# Autodesk Inventor assembly: Assembled
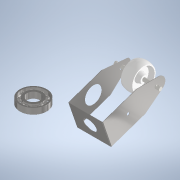
[picture p0: Inventor's stored thumbnail of the model, 180x180]
Saved by Autodesk Inventor 2020.3 (Build 243373000, 373)
## iProperties
Created: 2022-06-27
Part Number: Assembled
Document SubType Name: Assembly
Designer: 0x6f736f646f
Author: 0x6f736f646f
## Documents named in this file (5)
- C:\Users\Public\D\Desktop\mechanicalDesign\src\Assembled.iam
- C:\Users\Public\D\Desktop\mechanicalDesign\src\casterwheel.ipt
- C:\Users\Public\D\Desktop\mechanicalDesign\src\wheelshaftGenerated.ipt
- C:\Users\Public\D\Desktop\mechanicalDesign\src\Frame.ipt
- C:\Users\Public\D\Desktop\mechanicalDesign\src\BearingGenerated.iam
## Components (4 placed, 4 different names)
1. casterwheel:1 — Cylindrical:1
2. Shaft:1 — Cylindrical:1, Cylindrical:2
3. Frame:1 — Cylindrical:2
4. Bearing:1 [sub-assembly]
## Relationships (2: CylindricalJoint 2)
- Cylindrical:1: casterwheel:1 ↔ Shaft:1
- Cylindrical:2: Shaft:1 ↔ Frame:1
